# Autodesk Inventor assembly: Worm gear
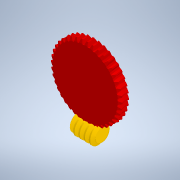
[picture p0: Inventor's stored thumbnail of the model, 180x180]
Saved by Autodesk Inventor 2021 (Build 250183000, 183)
## iProperties
Created: 2021-07-29
Part Number: Worm gear
Document SubType Name: Assembly
Designer: Shammy Haider
Author: Shammy Haider
## Documents named in this file (2)
- D:\Designing\Autodesk inventor\Worm gear.iam
- D:\Designing\Autodesk inventor\Worm gear\Design Accelerator\Worm Gears1.iam
## Components (1 placed, 1 different names)
1. Worm Gears:1 [sub-assembly] — Mate:1, Mate:3, Mate:4, Angle:1
## Relationships (4: Mate 3, Angle 1)
- Mate:1: Worm Gears:1
- Mate:3: Worm Gears:1
- Mate:4: Worm Gears:1
- Angle:1 (2815 deg): Worm Gears:1
